# Autodesk Inventor assembly: BumperCar
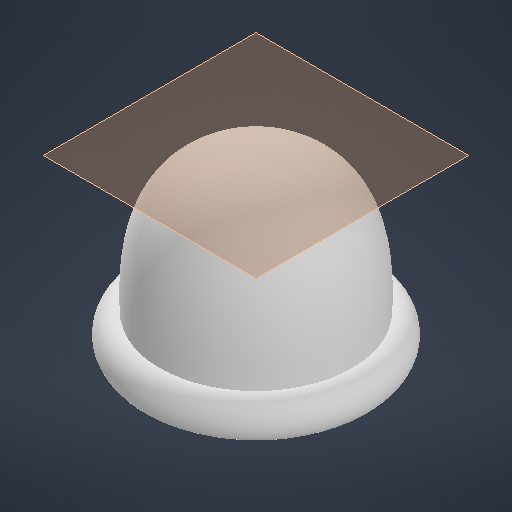
[picture p0: Inventor's stored thumbnail of the model, 512x512]
Saved by Autodesk Inventor 2026.1 (Build 301233000, 233)
## iProperties
Created: 2026-06-27
Part Number: BumperCar
Document SubType Name: Assembly
Designer: Kasi Pusuluri
Author: Kasi Pusuluri
## Documents named in this file (3)
- C:\Users\Kasi Pusuluri\Documents\Outpost 2026\BumperCar.iam
- C:\Users\Kasi Pusuluri\Documents\Outpost 2026\Bumper.ipt
- C:\Users\Kasi Pusuluri\Documents\Outpost 2026\BumperTop3.ipt
## Components (2 placed, 2 different names)
1. Bumper:1 — Rigid:1
2. BumperTop3:1 — Rigid:1
## Relationships (1: WeldJoint 1)
- Rigid:1 [WeldJoint]: Bumper:1 ↔ BumperTop3:1
